# Autodesk Inventor assembly: Out-PCB plus Connectors
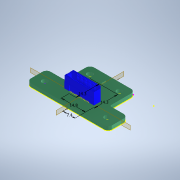
[picture p0: Inventor's stored thumbnail of the model, 180x180]
Saved by Autodesk Inventor 2021 (Build 250183000, 183)
## iProperties
Created: 2020-04-07
Part Number: Out-PCB plus Connectors
Document SubType Name: Assembly
Designer: jgray
Author: jgray
## Documents named in this file (4)
- M:\Printed Electronics\Gas Sensors\Prototypes\Prototype II -Cartridge Reader V2\Cartridge Interface V5 30-06-20\Out-PCB plus Connectors.iam
- M:\Printed Electronics\Gas Sensors\Prototypes\Prototype II -Cartridge Reader V2\Cartridge Interface V5 30-06-20\Digikey H125559CT-NDER8-30S-0.8SV-7H_TOP.iam
- M:\Printed Electronics\Gas Sensors\Prototypes\Prototype II -Cartridge Reader V2\Cartridge Interface V5 30-06-20\Out-facing Connector PCB.ipt
- M:\Printed Electronics\Gas Sensors\Prototypes\Prototype II -Cartridge Reader V2\Cartridge Interface V5 30-06-20\524653071.ipt
## Components (3 placed, 3 different names)
1. Digikey H125559CT-NDER8-30S-0.8SV-7H_TOP:1 [sub-assembly] — Angle:1, Tangent:1, Mate:1, Mate:2
2. Out-facing Connector PCB:1 — Angle:1, Tangent:1, Mate:1, Mate:2, Mate:3, Angle:2, Flush:1, Mate:5
3. 524653071:1 — Mate:4, Flush:2, Mate:5
## Relationships (10: Mate 5, Angle 2, Flush 2, Tangent 1)
- Angle:1 (180 deg): Digikey H125559CT-NDER8-30S-0.8SV-7H_TOP:1 ↔ Out-facing Connector PCB:1
- Tangent:1: Digikey H125559CT-NDER8-30S-0.8SV-7H_TOP:1 ↔ Out-facing Connector PCB:1
- Mate:1: Digikey H125559CT-NDER8-30S-0.8SV-7H_TOP:1 ↔ Out-facing Connector PCB:1
- Mate:2: Digikey H125559CT-NDER8-30S-0.8SV-7H_TOP:1 ↔ Out-facing Connector PCB:1
- Mate:3: Out-facing Connector PCB:1
- Angle:2 (0 deg): Out-facing Connector PCB:1
- Flush:1 (1.15 mm): Out-facing Connector PCB:1
- Mate:4: 524653071:1
- Flush:2: 524653071:1
- Mate:5: Out-facing Connector PCB:1 ↔ 524653071:1
